# Autodesk Inventor assembly: Motor Mount
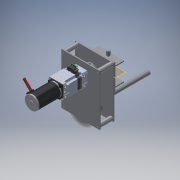
[picture p0: Inventor's stored thumbnail of the model, 180x180]
Saved by Autodesk Inventor 2019 (Build 230136000, 136)
## iProperties
Created: 2018-10-27
Part Number: Motor Mount
Document SubType Name: Assembly
Designer: olale
Mass: 511.238 g
Surface Area: 2454.31 cm^2
Volume: 511.238 cm^3
Density: 1 g/cm^3
Author: olale
## Documents named in this file (13)
- C:\Users\Swapnil\Desktop\ImportantThings\Robotics\Vanderbilt Robotics\2018-2019\FrameAndDrive\Motor Mount\Motor Mount.iam
- C:\Users\Swapnil\Desktop\ImportantThings\Robotics\Vanderbilt Robotics\2018-2019\FrameAndDrive\Motor Mount\Standoffs.ipt
- C:\Users\Swapnil\Desktop\ImportantThings\Robotics\Vanderbilt Robotics\2018-2019\FrameAndDrive\Right Angle Frame Mount.ipt
- C:\Users\Swapnil\Desktop\ImportantThings\Robotics\Vanderbilt Robotics\2018-2019\FrameAndDrive\DriveMotor\Drive Motor Assembly.iam
- C:\Users\Swapnil\Desktop\ImportantThings\Robotics\Vanderbilt Robotics\2018-2019\FrameAndDrive\Motor Mount\24 tooth sprocket\ONDRIVES_US_CORP_L50A-31DP-024.iam
- C:\Users\Swapnil\Desktop\ImportantThings\Robotics\Vanderbilt Robotics\2018-2019\FrameAndDrive\GearBoxFrontPlate.ipt
- C:\Users\Swapnil\Desktop\ImportantThings\Robotics\Vanderbilt Robotics\2018-2019\FrameAndDrive\Motor Mount\Standoffs_MIR.ipt
- C:\Users\Swapnil\Desktop\ImportantThings\Robotics\Vanderbilt Robotics\2018-2019\FrameAndDrive\GearBoxRearPlate.ipt
- C:\Users\Swapnil\Desktop\ImportantThings\Robotics\Vanderbilt Robotics\2018-2019\FrameAndDrive\Motor Mount\Standoffs_CPY.ipt
- C:\Users\Swapnil\Desktop\ImportantThings\Robotics\Vanderbilt Robotics\2018-2019\FrameAndDrive\Motor Mount\Standoffs_MIR_CPY.ipt
- C:\Users\Swapnil\Desktop\ImportantThings\Robotics\Vanderbilt Robotics\2018-2019\FrameAndDrive\Motor Mount\12 tooth sprocket\ONDRIVES_US_CORP_L50A-36DP-012.iam
- C:\Users\Swapnil\Desktop\ImportantThings\Robotics\Vanderbilt Robotics\2018-2019\FrameAndDrive\Shaft.ipt
- C:\Users\Swapnil\Desktop\ImportantThings\Robotics\Vanderbilt Robotics\2018-2019\FrameAndDrive\Pin.ipt
## Components (16 placed, 12 different names)
1. Right Angle Frame Mount:1 — Mate:16, Flush:1, Flush:2, Mate:43
2. Drive Motor Assembly:1 [sub-assembly] — Mate:32, Mate:33, Mate:35
3. ONDRIVES_US_CORP_L50A-31DP-024:1 [sub-assembly] — Mate:37, Mate:38
4. GearBoxFrontPlate:1 — Mate:16, Flush:1, Flush:2, Mate:17, Mate:18, Mate:19, Mate:20, Mate:30, Mate:39, Mate:40, Mate:41, Mate:42
5. Standoffs:1 — Mate:17, Mate:18, Mate:27, Mate:28
6. Standoffs:2 — Mate:19, Mate:20, Mate:25, Mate:26
7. Standoffs_MIR:1 — Mate:23, Mate:24, Mate:39, Mate:40
8. Standoffs_MIR:2 — Mate:21, Mate:22, Mate:41, Mate:42
9. GearBoxRearPlate:1 — Mate:29, Mate:30, Mate:31, Mate:32, Mate:33, Mate:34, Mate:36, Flush:3, Mate:38
10. Standoffs_CPY:1 — Mate:27, Mate:28, Mate:29, Mate:31
11. Standoffs_CPY:2 — Mate:25, Mate:26
12. Standoffs_MIR_CPY:1 — Mate:23, Mate:24
13. Standoffs_MIR_CPY:2 — Mate:21, Mate:22
14. ONDRIVES_US_CORP_L50A-36DP-012:1 [sub-assembly] — Mate:34, Mate:35
15. Shaft:1 — Mate:36, Flush:3, Mate:37
16. Pin:1 — Mate:43
## Relationships (31: Mate 28, Flush 3)
- Mate:16: Right Angle Frame Mount:1 ↔ GearBoxFrontPlate:1
- Flush:1: Right Angle Frame Mount:1 ↔ GearBoxFrontPlate:1
- Flush:2: Right Angle Frame Mount:1 ↔ GearBoxFrontPlate:1
- Mate:17: GearBoxFrontPlate:1 ↔ Standoffs:1
- Mate:18: GearBoxFrontPlate:1 ↔ Standoffs:1
- Mate:19: GearBoxFrontPlate:1 ↔ Standoffs:2
- Mate:20: GearBoxFrontPlate:1 ↔ Standoffs:2
- Mate:21: Standoffs_MIR:2 ↔ Standoffs_MIR_CPY:2
- Mate:22: Standoffs_MIR:2 ↔ Standoffs_MIR_CPY:2
- Mate:23: Standoffs_MIR:1 ↔ Standoffs_MIR_CPY:1
- Mate:24: Standoffs_MIR:1 ↔ Standoffs_MIR_CPY:1
- Mate:25: Standoffs:2 ↔ Standoffs_CPY:2
- Mate:26: Standoffs:2 ↔ Standoffs_CPY:2
- Mate:27: Standoffs:1 ↔ Standoffs_CPY:1
- Mate:28: Standoffs:1 ↔ Standoffs_CPY:1
- Mate:29: GearBoxRearPlate:1 ↔ Standoffs_CPY:1
- Mate:30: GearBoxFrontPlate:1 ↔ GearBoxRearPlate:1
- Mate:31: GearBoxRearPlate:1 ↔ Standoffs_CPY:1
- Mate:32: Drive Motor Assembly:1 ↔ GearBoxRearPlate:1
- Mate:33: Drive Motor Assembly:1 ↔ GearBoxRearPlate:1
- Mate:34: GearBoxRearPlate:1 ↔ ONDRIVES_US_CORP_L50A-36DP-012:1
- Mate:35: Drive Motor Assembly:1 ↔ ONDRIVES_US_CORP_L50A-36DP-012:1
- Mate:36: GearBoxRearPlate:1 ↔ Shaft:1
- Flush:3: GearBoxRearPlate:1 ↔ Shaft:1
- Mate:37: ONDRIVES_US_CORP_L50A-31DP-024:1 ↔ Shaft:1
- Mate:38: ONDRIVES_US_CORP_L50A-31DP-024:1 ↔ GearBoxRearPlate:1
- Mate:39: GearBoxFrontPlate:1 ↔ Standoffs_MIR:1
- Mate:40: GearBoxFrontPlate:1 ↔ Standoffs_MIR:1
- Mate:41: GearBoxFrontPlate:1 ↔ Standoffs_MIR:2
- Mate:42: GearBoxFrontPlate:1 ↔ Standoffs_MIR:2
- Mate:43 (-50.8 mm): Right Angle Frame Mount:1 ↔ Pin:1
